# Autodesk Inventor assembly: intake2
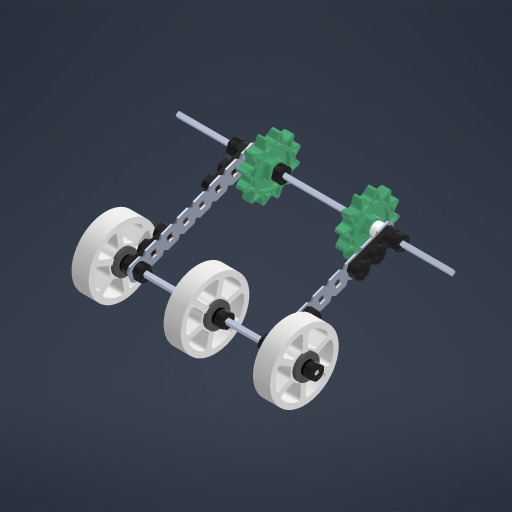
[picture p0: Inventor's stored thumbnail of the model, 512x512]
Saved by Autodesk Inventor 2023 (Build 270158000, 158)
## iProperties
Created: 2023-03-02
Part Number: intake2
Document SubType Name: Assembly
Designer: Windows Macbook
Author: Windows Macbook
## Documents named in this file (12)
- C:\Users\Windows Macbook\Desktop\VRC-SPIN-UP\Inventor\Assembly\Pre Worlds\intake2.iam
- C:\Users\Windows Macbook\Desktop\VRC-SPIN-UP\Inventor\Motion\Wheels\Flex Wheels\2 Flex, LS.iam
- C:\Users\Windows Macbook\Desktop\VRC-SPIN-UP\Inventor\Motion\Sprockets\9P Sprocket\9P 12T Sprocket, Square.iam
- C:\Users\Windows Macbook\Desktop\VRC-SPIN-UP\Inventor\Motion\Sprockets\9P Sprocket.iam
- C:\Users\Windows Macbook\Desktop\VRC-SPIN-UP\Inventor\Motion\Shaft LS\Shaft LS\Shaft LS 8.0.ipt
- C:\Users\Windows Macbook\Desktop\VRC-SPIN-UP\Inventor\Motion\Shaft LS\Shaft LS.ipt
- C:\Users\Windows Macbook\Desktop\VRC-SPIN-UP\Inventor\Structure\Plate\Steel\Steel Plate 1x8.ipt
- C:\Users\Windows Macbook\Desktop\VRC-SPIN-UP\Inventor\Motion\Shaft LS\Bearing Flat.ipt
- C:\Users\Windows Macbook\Desktop\VRC-SPIN-UP\Inventor\Motion\Spacers\Spacer Nylon .313 OD\NSpacer .313 OD x .250.ipt
- C:\Users\Windows Macbook\Desktop\VRC-SPIN-UP\Inventor\Motion\Spacers\Spacer Nylon .313 OD.ipt
- C:\Users\Windows Macbook\Desktop\VRC-SPIN-UP\Inventor\Motion\Shaft LS\Shaft Collar Rubber.ipt
- C:\Users\Windows Macbook\Desktop\VRC-SPIN-UP\Inventor\Motion\Shaft LS\Shaft LS\Shaft LS 6.5.ipt
## Components (25 placed, 8 different names)
1. 2 Flex, LS:1 [sub-assembly]
2. 9P 12T Sprocket, Square:1 [sub-assembly]
3. 9P 12T Sprocket, Square:2 [sub-assembly]
4. 2 Flex, LS:2 [sub-assembly]
5. Shaft LS 8.0:1
6. Steel Plate 1x8:1
7. Bearing Flat:1
8. NSpacer .313 OD x .250:1
9. Bearing Flat:2
10. 2 Flex, LS:3 [sub-assembly]
11. Steel Plate 1x8:2
12. Bearing Flat:3
13. NSpacer .313 OD x .250:2
14. Bearing Flat:4
15. Shaft Collar Rubber:1
16. Shaft Collar Rubber:2
17. Shaft Collar Rubber:3
18. Shaft Collar Rubber:4
19. Shaft Collar Rubber:5
20. Shaft Collar Rubber:6
21. Shaft Collar Rubber:7
22. Shaft Collar Rubber:8
23. Shaft Collar Rubber:9
24. Shaft Collar Rubber:10
25. Shaft LS 6.5:2
## Relationships (28: Insert 25, CylindricalJoint 2, Flush 1)
- [Insert]: Steel Plate 1x8:1 ↔ Bearing Flat:1
- [Insert]: Steel Plate 1x8:1 ↔ Bearing Flat:1
- [Insert]: 9P 12T Sprocket, Square:2 ↔ NSpacer .313 OD x .250:1
- [Insert]: Steel Plate 1x8:1 ↔ NSpacer .313 OD x .250:1
- [Insert]: Steel Plate 1x8:1 ↔ Bearing Flat:2
- [Insert]: Steel Plate 1x8:1 ↔ Bearing Flat:2
- [Insert]: 2 Flex, LS:1 ↔ Bearing Flat:2
- [Insert]: Steel Plate 1x8:2 ↔ Bearing Flat:3
- [Insert]: Steel Plate 1x8:2 ↔ Bearing Flat:3
- [Insert]: Steel Plate 1x8:2 ↔ NSpacer .313 OD x .250:2
- [Insert]: Steel Plate 1x8:2 ↔ Bearing Flat:4
- [Insert]: Steel Plate 1x8:2 ↔ Bearing Flat:4
- [Insert]: 2 Flex, LS:3 ↔ Bearing Flat:4
- [Insert]: 9P 12T Sprocket, Square:1 ↔ NSpacer .313 OD x .250:2
- [Insert] (0.889 mm): Bearing Flat:1 ↔ Shaft Collar Rubber:2
- [Insert] (0.889 mm): 9P 12T Sprocket, Square:2 ↔ Shaft Collar Rubber:1
- [Insert] (0.889 mm): Bearing Flat:3 ↔ Shaft Collar Rubber:3
- [Insert] (0.889 mm): 9P 12T Sprocket, Square:1 ↔ Shaft Collar Rubber:4
- [Insert] (40.64 mm): 2 Flex, LS:2 ↔ Steel Plate 1x8:2
- [Insert] (0.889 mm): 2 Flex, LS:2 ↔ Shaft Collar Rubber:5
- [Insert] (0.889 mm): 2 Flex, LS:1 ↔ Shaft Collar Rubber:6
- [Insert] (0.889 mm): Steel Plate 1x8:2 ↔ Shaft Collar Rubber:7
- [Insert] (0.889 mm): 2 Flex, LS:3 ↔ Shaft Collar Rubber:10
- [Insert] (0.889 mm): 2 Flex, LS:2 ↔ Shaft Collar Rubber:9
- [Insert] (0.889 mm): Steel Plate 1x8:1 ↔ Shaft Collar Rubber:8
- [Flush]: Shaft Collar Rubber:6 ↔ Shaft LS 6.5:2
- [CylindricalJoint]: Shaft Collar Rubber:6 ↔ Shaft LS 6.5:2
- [CylindricalJoint]: Shaft Collar Rubber:10 ↔ Shaft LS 6.5:2
## Named parameters: d16_d26 = 0 mm, d17_d27 = 0 mm, d18_d28 = 0 mm, d19_d29 = 0 mm, d33_d26 = 0 mm, d34_d27 = 0 mm, d35_d29 = 0 mm, d36_d30 = 0 mm, d37_d31 = 0 mm, d38_d32 = 0 mm
